# Autodesk Inventor assembly: ToughBoxMiniWith2CimMotors
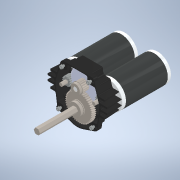
[picture p0: Inventor's stored thumbnail of the model, 180x180]
Saved by Autodesk Inventor 2020.2 (Build 242310000, 310)
## iProperties
Created: 2020-01-26
Part Number: ToughBoxMiniWith2CimMotors
Document SubType Name: Assembly
Designer: robst
Author: robst
## Documents named in this file (3)
- C:\git\CAD-Development\robSteele\2020CompetitionRobot\ToughBoxMiniWith2CimMotors.iam
- C:\git\CAD-Development\robSteele\2020CompetitionRobot\am-2598_107 2016 KOP Toughbox Mini.iam
- C:\git\CAD-Development\robSteele\2020CompetitionRobot\CIM Motor SW.ipt
## Components (3 placed, 2 different names)
1. am-2598_107 2016 KOP Toughbox Mini:1 [sub-assembly] — Insert:1, Insert:2, Insert:3, Insert:4
2. CIM Motor SW:1 — Insert:1, Insert:2
3. CIM Motor SW:2 — Insert:3, Insert:4
## Relationships (4: Insert 4)
- Insert:1: am-2598_107 2016 KOP Toughbox Mini:1 ↔ CIM Motor SW:1
- Insert:2: am-2598_107 2016 KOP Toughbox Mini:1 ↔ CIM Motor SW:1
- Insert:3: am-2598_107 2016 KOP Toughbox Mini:1 ↔ CIM Motor SW:2
- Insert:4: am-2598_107 2016 KOP Toughbox Mini:1 ↔ CIM Motor SW:2
